# Autodesk Inventor assembly: DGB_000_DriveGearBox_MIR
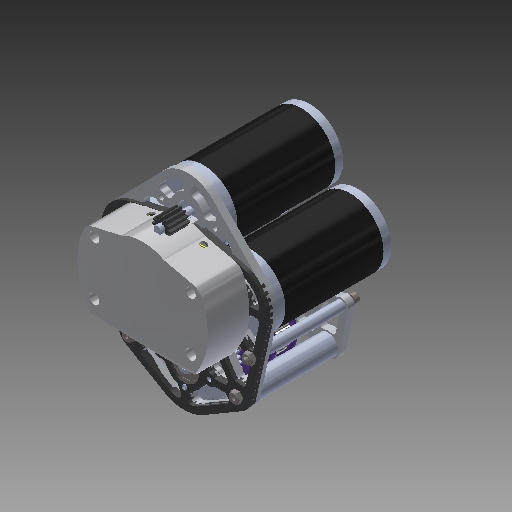
[picture p0: Inventor's stored thumbnail of the model, 512x512]
Saved by Autodesk Inventor 2018.3 (Build 223284000, 284)
## iProperties
Created: 2020-01-12
Part Number: DGB_000_DriveGearBox_MIR
Document SubType Name: Assembly
Designer: Alex
Mass: 1560.09 g
Surface Area: 3977.44 cm^2
Volume: 1551.03 cm^3
Density: 1.00584 g/cm^3
Author: user
## Documents named in this file (6)
- C:\Users\22turnmaxw\Documents\GrabCAD\Infinite Recharge 2020\Build season\DGB_000_DriveGearBox_MIR.iam
- C:\Users\22turnmaxw\Documents\GrabCAD\Infinite Recharge 2020\Brainstorming\WCP-0155 Rev1 - WCP 3 Motor Flipped Gearbox (SS)2018_MIR.iam
- C:\Users\22turnmaxw\Documents\GrabCAD\Infinite Recharge 2020\Build season\DGB_002_NewCover_MIR.ipt
- C:\Users\22turnmaxw\Documents\GrabCAD\Infinite Recharge 2020\Build season\CHA_006_DrivePulleyAssembly_MIR.iam
- C:\Users\22turnmaxw\Documents\GrabCAD\Infinite Recharge 2020\Build season\DGB_003_1.375HexSpacer_MIR.ipt
- C:\Users\22turnmaxw\Documents\GrabCAD\Infinite Recharge 2020\Build season\DGB_004_OutputWheelSpacer_MIR.ipt
## Components (5 placed, 5 different names)
1. WCP-0155 Rev1 - WCP 3 Motor Flipped Gearbox (SS)2018_MIR:1 [sub-assembly] — Mate:6, Mate:5, Mate:4, Mate:9, Mate:8, Mate:7, Mate:12, Mate:11, Mate:14, Mate:13
2. DGB_002_NewCover_MIR:1 — Mate:6, Mate:5, Mate:4
3. CHA_006_DrivePulleyAssembly_MIR:1 [sub-assembly] — Mate:9, Mate:8, Mate:7, Mate:10
4. DGB_003_1.375HexSpacer_MIR:1 — Mate:12, Mate:11, Mate:10, Flush:1
5. DGB_004_OutputWheelSpacer_MIR:1 — Flush:1, Mate:14, Mate:13
## Relationships (12: Mate 11, Flush 1)
- Mate:6: WCP-0155 Rev1 - WCP 3 Motor Flipped Gearbox (SS)2018_MIR:1 ↔ DGB_002_NewCover_MIR:1
- Mate:5: WCP-0155 Rev1 - WCP 3 Motor Flipped Gearbox (SS)2018_MIR:1 ↔ DGB_002_NewCover_MIR:1
- Mate:4: WCP-0155 Rev1 - WCP 3 Motor Flipped Gearbox (SS)2018_MIR:1 ↔ DGB_002_NewCover_MIR:1
- Mate:9 (3.7846 mm): WCP-0155 Rev1 - WCP 3 Motor Flipped Gearbox (SS)2018_MIR:1 ↔ CHA_006_DrivePulleyAssembly_MIR:1
- Mate:8: WCP-0155 Rev1 - WCP 3 Motor Flipped Gearbox (SS)2018_MIR:1 ↔ CHA_006_DrivePulleyAssembly_MIR:1
- Mate:7: WCP-0155 Rev1 - WCP 3 Motor Flipped Gearbox (SS)2018_MIR:1 ↔ CHA_006_DrivePulleyAssembly_MIR:1
- Mate:12: WCP-0155 Rev1 - WCP 3 Motor Flipped Gearbox (SS)2018_MIR:1 ↔ DGB_003_1.375HexSpacer_MIR:1
- Mate:11: WCP-0155 Rev1 - WCP 3 Motor Flipped Gearbox (SS)2018_MIR:1 ↔ DGB_003_1.375HexSpacer_MIR:1
- Mate:10: CHA_006_DrivePulleyAssembly_MIR:1 ↔ DGB_003_1.375HexSpacer_MIR:1
- Flush:1 (12.827 mm): DGB_003_1.375HexSpacer_MIR:1 ↔ DGB_004_OutputWheelSpacer_MIR:1
- Mate:14: WCP-0155 Rev1 - WCP 3 Motor Flipped Gearbox (SS)2018_MIR:1 ↔ DGB_004_OutputWheelSpacer_MIR:1
- Mate:13: WCP-0155 Rev1 - WCP 3 Motor Flipped Gearbox (SS)2018_MIR:1 ↔ DGB_004_OutputWheelSpacer_MIR:1
